# Autodesk Inventor assembly: OmniWheel
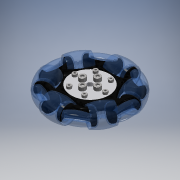
[picture p0: Inventor's stored thumbnail of the model, 180x180]
Saved by Autodesk Inventor 2018.3 (Build 223284000, 284)
## iProperties
Created: 2018-08-15
Part Number: OmniWheel
Material: Generisch
Document SubType Name: Assembly
Designer: JochenAlt
Author: JochenAlt
## Documents named in this file (6)
- D:\Projects\FlowerPot\CAD\OmniWheel.iam
- D:\Projects\FlowerPot\CAD\OmniWheel.ipt
- D:\Projects\FlowerPot\CAD\Mounting Hub.ipt
- C:\Users\JochenAlt\Documents\Inventor\Content Center Files\R2018\de-DE\DIN 912\DIN 912 - M3 x 0,5 x 8 x 6,75.ipt
- C:\Users\JochenAlt\Documents\Inventor\Content Center Files\R2018\de-DE\DIN 912\DIN 912 - M2 x 0,4 x 8 x 7.ipt
- C:\Users\JochenAlt\Documents\Inventor\Content Center Files\R2018\de-DE\DIN 934\DIN 934 - M2 x 0,4.ipt
## Components (18 placed, 5 different names)
1. OmniWheel:1 — Passend:1, Passend:2, Einfügen:1, Einfügen:2, Einfügen:3, Einfügen:4, Einfügen:5, Einfügen:6, Einfügen:7, Einfügen:8, Einfügen:9, Einfügen:10, Passend:4, Passend:6, Passend:8, Passend:10, Passend:12, Passend:14
2. Mounting Hub:1 — Passend:1, Passend:2
3. DIN 912 - ersetzt durch DIN EN ISO 4762 M3 x 8:1 — Einfügen:1
4. DIN 912 - ersetzt durch DIN EN ISO 4762 M3 x 8:2 — Einfügen:2
5. DIN 912 - ersetzt durch DIN EN ISO 4762 M3 x 8:3 — Einfügen:3
6. DIN 912 - ersetzt durch DIN EN ISO 4762 M3 x 8:4 — Einfügen:4
7. DIN 912 - ersetzt durch DIN EN ISO 4762 M2 x 8:1 — Einfügen:5, Passend:13
8. DIN 912 - ersetzt durch DIN EN ISO 4762 M2 x 8:2 — Einfügen:6, Passend:9
9. DIN 912 - ersetzt durch DIN EN ISO 4762 M2 x 8:3 — Einfügen:7, Passend:7
10. DIN 912 - ersetzt durch DIN EN ISO 4762 M2 x 8:4 — Einfügen:8, Passend:5
11. DIN 912 - ersetzt durch DIN EN ISO 4762 M2 x 8:5 — Einfügen:9, Passend:11
12. DIN 912 - ersetzt durch DIN EN ISO 4762 M2 x 8:6 — Einfügen:10, Passend:3
13. DIN 934 - ersetzt durch DIN EN 24032/28673/28674 M2:1 — Passend:3, Passend:4
14. DIN 934 - ersetzt durch DIN EN 24032/28673/28674 M2:2 — Passend:5, Passend:6
15. DIN 934 - ersetzt durch DIN EN 24032/28673/28674 M2:3 — Passend:7, Passend:8
16. DIN 934 - ersetzt durch DIN EN 24032/28673/28674 M2:4 — Passend:9, Passend:10
17. DIN 934 - ersetzt durch DIN EN 24032/28673/28674 M2:5 — Passend:11, Passend:12
18. DIN 934 - ersetzt durch DIN EN 24032/28673/28674 M2:6 — Passend:13, Passend:14
## Relationships (24: Mate 14, Insert 10)
- Passend:1 [Mate]: OmniWheel:1 ↔ Mounting Hub:1
- Passend:2 [Mate]: OmniWheel:1 ↔ Mounting Hub:1
- Einfügen:1 [Insert]: OmniWheel:1 ↔ DIN 912 - ersetzt durch DIN EN ISO 4762 M3 x 8:1
- Einfügen:2 [Insert]: OmniWheel:1 ↔ DIN 912 - ersetzt durch DIN EN ISO 4762 M3 x 8:2
- Einfügen:3 [Insert]: OmniWheel:1 ↔ DIN 912 - ersetzt durch DIN EN ISO 4762 M3 x 8:3
- Einfügen:4 [Insert]: OmniWheel:1 ↔ DIN 912 - ersetzt durch DIN EN ISO 4762 M3 x 8:4
- Einfügen:5 [Insert]: OmniWheel:1 ↔ DIN 912 - ersetzt durch DIN EN ISO 4762 M2 x 8:1
- Einfügen:6 [Insert]: OmniWheel:1 ↔ DIN 912 - ersetzt durch DIN EN ISO 4762 M2 x 8:2
- Einfügen:7 [Insert]: OmniWheel:1 ↔ DIN 912 - ersetzt durch DIN EN ISO 4762 M2 x 8:3
- Einfügen:8 [Insert]: OmniWheel:1 ↔ DIN 912 - ersetzt durch DIN EN ISO 4762 M2 x 8:4
- Einfügen:9 [Insert]: OmniWheel:1 ↔ DIN 912 - ersetzt durch DIN EN ISO 4762 M2 x 8:5
- Einfügen:10 [Insert]: OmniWheel:1 ↔ DIN 912 - ersetzt durch DIN EN ISO 4762 M2 x 8:6
- Passend:3 [Mate]: DIN 912 - ersetzt durch DIN EN ISO 4762 M2 x 8:6 ↔ DIN 934 - ersetzt durch DIN EN 24032/28673/28674 M2:1
- Passend:4 [Mate]: OmniWheel:1 ↔ DIN 934 - ersetzt durch DIN EN 24032/28673/28674 M2:1
- Passend:5 [Mate]: DIN 912 - ersetzt durch DIN EN ISO 4762 M2 x 8:4 ↔ DIN 934 - ersetzt durch DIN EN 24032/28673/28674 M2:2
- Passend:6 [Mate]: OmniWheel:1 ↔ DIN 934 - ersetzt durch DIN EN 24032/28673/28674 M2:2
- Passend:7 [Mate]: DIN 912 - ersetzt durch DIN EN ISO 4762 M2 x 8:3 ↔ DIN 934 - ersetzt durch DIN EN 24032/28673/28674 M2:3
- Passend:8 [Mate]: OmniWheel:1 ↔ DIN 934 - ersetzt durch DIN EN 24032/28673/28674 M2:3
- Passend:9 [Mate]: DIN 912 - ersetzt durch DIN EN ISO 4762 M2 x 8:2 ↔ DIN 934 - ersetzt durch DIN EN 24032/28673/28674 M2:4
- Passend:10 [Mate]: OmniWheel:1 ↔ DIN 934 - ersetzt durch DIN EN 24032/28673/28674 M2:4
- Passend:11 [Mate]: DIN 912 - ersetzt durch DIN EN ISO 4762 M2 x 8:5 ↔ DIN 934 - ersetzt durch DIN EN 24032/28673/28674 M2:5
- Passend:12 [Mate]: OmniWheel:1 ↔ DIN 934 - ersetzt durch DIN EN 24032/28673/28674 M2:5
- Passend:13 [Mate]: DIN 912 - ersetzt durch DIN EN ISO 4762 M2 x 8:1 ↔ DIN 934 - ersetzt durch DIN EN 24032/28673/28674 M2:6
- Passend:14 [Mate]: OmniWheel:1 ↔ DIN 934 - ersetzt durch DIN EN 24032/28673/28674 M2:6
